# Autodesk Inventor assembly: Front_Kicker_Assembly
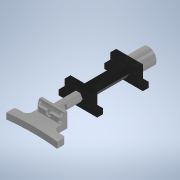
[picture p0: Inventor's stored thumbnail of the model, 180x180]
Saved by Autodesk Inventor 2020 (Build 240168000, 168)
## iProperties
Created: 2019-06-09
Part Number: Front_Kicker_Assembly
Document SubType Name: Assembly
Designer: Martins
Author: Martins
## Documents named in this file (4)
- C:\Users\victo\Documents\ssl-mechanics\V2.0(RoboCup2019)\Inventor\Kicker\Front_Kicker_Assembly.iam
- C:\Users\victo\Documents\ssl-mechanics\V2.0(RoboCup2019)\Inventor\Kicker\Front_Kicker_Coil.ipt
- C:\Users\victo\Documents\ssl-mechanics\V2.0(RoboCup2019)\Inventor\Kicker\ThreadHolder_Kicker.ipt
- C:\Users\victo\Documents\ssl-mechanics\V2.0(RoboCup2019)\Inventor\Kicker\Front_Kicker.ipt
## Components (3 placed, 3 different names)
1. Front_Kicker_Coil:1 — Slider:1
2. ThreadHolder_Kicker:1 — Slider:1, Rigid:1
3. Front_Kicker:1 — Rigid:1
## Relationships (2: TranslationJoint 1, WeldJoint 1)
- Slider:1 [TranslationJoint] (0.2 mm): Front_Kicker_Coil:1 ↔ ThreadHolder_Kicker:1
- Rigid:1 [WeldJoint] (0.2 mm): ThreadHolder_Kicker:1 ↔ Front_Kicker:1
